# Autodesk Inventor assembly: Montagem1.Trechos de tubos e tubulações
(part 2 of 2)
## Documents named in this file (2)
- C:\Users\Olá\programacao\nasa\drone\Montagem1\AIP\Tubos e tubulações\Montagem1.Trechos de tubos e tubulações.iam
- C:\Users\Olá\programacao\nasa\drone\Montagem1\AIP\Tubos e tubulações\Trecho01\Montagem1.Trecho01.iam
## Components (1 placed, 1 different names)
1. Trecho 01 [sub-assembly]
